# Autodesk Inventor assembly: パネル型スカラアームMISUMIアルミフレーム作成Ver
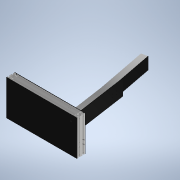
[picture p0: Inventor's stored thumbnail of the model, 180x180]
Saved by Autodesk Inventor 2022 (Build 260153000, 153)
## iProperties
Created: 2022-12-05
Part Number: パネル型スカラアームMISUMIアルミフレーム作成Ver
Document SubType Name: Assembly
Designer: tdn82
Author: tdn82
## Documents named in this file (20)
- C:\Users\tdn82\OneDrive\ドキュメント\Inventor\卒業研究パネル型スカラアーム\GrabCAD\panel-type-scalar-arm\パネル型スカラアーム\パネル型スカラアームMISUMIアルミフレーム作成Ver.iam
- C:\Users\tdn82\OneDrive\ドキュメント\Inventor\卒業研究パネル型スカラアーム\GrabCAD\panel-type-scalar-arm\パネル型スカラアーム\HFSF5-2040-180-LWH-RWH.ipt
- C:\Users\tdn82\OneDrive\ドキュメント\Inventor\卒業研究パネル型スカラアーム\GrabCAD\panel-type-scalar-arm\パネル型スカラアーム\HFSF5-2040-320-TPW.ipt
- C:\Users\tdn82\OneDrive\ドキュメント\Inventor\卒業研究パネル型スカラアーム\GrabCAD\panel-type-scalar-arm\パネル型スカラアーム\後ろカバー.ipt
- C:\Users\tdn82\OneDrive\ドキュメント\Inventor\卒業研究パネル型スカラアーム\GrabCAD\panel-type-scalar-arm\パネル型スカラアーム\サーボモータ固定用１軸目.ipt
- C:\Users\tdn82\OneDrive\ドキュメント\Inventor\卒業研究パネル型スカラアーム\GrabCAD\panel-type-scalar-arm\パネル型スカラアーム\サーボモータB3M-SC-1170-AB3M1100_scale.ipt
- C:\Users\tdn82\OneDrive\ドキュメント\Inventor\卒業研究パネル型スカラアーム\GrabCAD\panel-type-scalar-arm\パネル型スカラアーム\サーボ固定パーツ３Dプリンタ出力実験\サーボモータ固定用２軸目3mm改.ipt
- C:\Users\tdn82\OneDrive\ドキュメント\Inventor\卒業研究パネル型スカラアーム\GrabCAD\panel-type-scalar-arm\パネル型スカラアーム\横長2ndフラットバー上 アルミフレーム用.ipt
- C:\Users\tdn82\OneDrive\ドキュメント\Inventor\卒業研究パネル型スカラアーム\GrabCAD\panel-type-scalar-arm\パネル型スカラアーム\前カバー中盤左アーム固定.ipt
- C:\Users\tdn82\OneDrive\ドキュメント\Inventor\卒業研究パネル型スカラアーム\GrabCAD\panel-type-scalar-arm\パネル型スカラアーム\アルミフリーホーン02137_AluminumFreeHornWithBearing_B3M_6000.ipt
- C:\Users\tdn82\OneDrive\ドキュメント\Inventor\卒業研究パネル型スカラアーム\GrabCAD\panel-type-scalar-arm\パネル型スカラアーム\横長3rdフラットバー下.ipt
- C:\Users\tdn82\OneDrive\ドキュメント\Inventor\卒業研究パネル型スカラアーム\GrabCAD\panel-type-scalar-arm\パネル型スカラアーム\横長2ndフラットバー下 アルミフレーム用.ipt
- C:\Users\tdn82\OneDrive\ドキュメント\Inventor\卒業研究パネル型スカラアーム\GrabCAD\panel-type-scalar-arm\パネル型スカラアーム\前カバー中段右.ipt
- C:\Users\tdn82\OneDrive\ドキュメント\Inventor\卒業研究パネル型スカラアーム\GrabCAD\panel-type-scalar-arm\パネル型スカラアーム\前上カバーサーボ隠し.ipt
- C:\Users\tdn82\OneDrive\ドキュメント\Inventor\卒業研究パネル型スカラアーム\GrabCAD\panel-type-scalar-arm\パネル型スカラアーム\前下カバーサーボ隠し.ipt
- C:\Users\tdn82\OneDrive\ドキュメント\Inventor\卒業研究パネル型スカラアーム\GrabCAD\panel-type-scalar-arm\パネル型スカラアーム\ベアリング.ipt
- C:\Users\tdn82\OneDrive\ドキュメント\Inventor\卒業研究パネル型スカラアーム\GrabCAD\panel-type-scalar-arm\パネル型スカラアーム\シャフト.ipt
- C:\Users\tdn82\OneDrive\ドキュメント\Inventor\卒業研究パネル型スカラアーム\GrabCAD\panel-type-scalar-arm\パネル型スカラアーム\シャフトカラー.ipt
- C:\Users\tdn82\OneDrive\ドキュメント\Inventor\卒業研究パネル型スカラアーム\GrabCAD\panel-type-scalar-arm\パネル型スカラアーム\三段目アクリル板.ipt
- C:\Users\tdn82\OneDrive\ドキュメント\Inventor\卒業研究パネル型スカラアーム\GrabCAD\panel-type-scalar-arm\パネル型スカラアーム\シャフトカラー.iam
## Components (23 placed, 18 different names)
1. HFSF5-2040-180-LWH-RWH:1 — 挿入:6, 挿入:8, 挿入:33, 挿入:34
2. HFSF5-2040-180-LWH-RWH:2 — 挿入:5, 挿入:7, メイト:4, フラッシュ:1, メイト:12, メイト:14, メイト:26, フラッシュ:4
3. HFSF5-2040-320-TPW:1 — 挿入:5, 挿入:6, 挿入:7, 挿入:8, メイト:1, メイト:5, メイト:13
4. HFSF5-2040-320-TPW:2 — 挿入:33, 挿入:34
5. 後ろカバー:1 — メイト:1, メイト:26, フラッシュ:4
6. サーボモータ固定用１軸目:1 — 挿入:11, 挿入:12, 挿入:13, メイト:4, フラッシュ:1
7. サーボモータB3M-SC-1170-AB3M1100_scale:1 — 挿入:11, 挿入:12, 挿入:13, メイト:5, 挿入:14
8. サーボモータ固定用２軸目3mm改:1 — 挿入:15, 挿入:16, 挿入:18, 挿入:19
9. 横長2ndフラットバー上 アルミフレーム用:1 — 挿入:14, メイト:7, フラッシュ:3, メイト:19
10. 前カバー中盤左アーム固定:1 — メイト:7, 挿入:15, 挿入:16, 挿入:23, 挿入:24, フラッシュ:3, メイト:19
11. サーボモータB3M-SC-1170-AB3M1100_scale:2 — 挿入:17, 挿入:18, 挿入:19, メイト:22, 挿入:32
12. アルミフリーホーン02137_AluminumFreeHornWithBearing_B3M_6000:1 — 挿入:17, 挿入:30, 挿入:31
13. 横長3rdフラットバー下:1 — フラッシュ:2, メイト:22, 挿入:32, メイト:25
14. 横長3rdフラットバー下:2 — フラッシュ:2, 挿入:30, 挿入:31, メイト:23, メイト:24
15. 横長2ndフラットバー下 アルミフレーム用:1 — 挿入:23, 挿入:24, 挿入:26
16. 前カバー中段右:1 — メイト:12, メイト:15, メイト:16, メイト:17, メイト:18
17. 前上カバーサーボ隠し:1 — メイト:13, メイト:14, メイト:15, メイト:16
18. 前下カバーサーボ隠し:1 — メイト:17, メイト:18
19. ベアリング:1 — 挿入:26, 挿入:35
20. シャフト:1 — 挿入:36
21. シャフトカラー:2 — 挿入:35, 挿入:36, 挿入:37
22. 三段目アクリル板:1 — メイト:23, メイト:24, メイト:25
23. シャフトカラー:3 [sub-assembly] — 挿入:37
## Relationships (45: Insert 24, Mate 17, Flush 4)
- 挿入:5 [Insert]: HFSF5-2040-180-LWH-RWH:2 ↔ HFSF5-2040-320-TPW:1
- 挿入:6 [Insert]: HFSF5-2040-180-LWH-RWH:1 ↔ HFSF5-2040-320-TPW:1
- 挿入:7 [Insert]: HFSF5-2040-180-LWH-RWH:2 ↔ HFSF5-2040-320-TPW:1
- 挿入:8 [Insert]: HFSF5-2040-180-LWH-RWH:1 ↔ HFSF5-2040-320-TPW:1
- メイト:1 [Mate]: HFSF5-2040-320-TPW:1 ↔ 後ろカバー:1
- 挿入:11 [Insert]: サーボモータ固定用１軸目:1 ↔ サーボモータB3M-SC-1170-AB3M1100_scale:1
- 挿入:12 [Insert]: サーボモータ固定用１軸目:1 ↔ サーボモータB3M-SC-1170-AB3M1100_scale:1
- 挿入:13 [Insert]: サーボモータ固定用１軸目:1 ↔ サーボモータB3M-SC-1170-AB3M1100_scale:1
- メイト:4 [Mate]: HFSF5-2040-180-LWH-RWH:2 ↔ サーボモータ固定用１軸目:1
- フラッシュ:1 [Flush]: HFSF5-2040-180-LWH-RWH:2 ↔ サーボモータ固定用１軸目:1
- メイト:5 [Mate] (0.5 mm): HFSF5-2040-320-TPW:1 ↔ サーボモータB3M-SC-1170-AB3M1100_scale:1
- 挿入:14 [Insert]: サーボモータB3M-SC-1170-AB3M1100_scale:1 ↔ 横長2ndフラットバー上 アルミフレーム用:1
- メイト:7 [Mate]: 横長2ndフラットバー上 アルミフレーム用:1 ↔ 前カバー中盤左アーム固定:1
- 挿入:15 [Insert]: サーボモータ固定用２軸目3mm改:1 ↔ 前カバー中盤左アーム固定:1
- 挿入:16 [Insert]: サーボモータ固定用２軸目3mm改:1 ↔ 前カバー中盤左アーム固定:1
- 挿入:17 [Insert]: サーボモータB3M-SC-1170-AB3M1100_scale:2 ↔ アルミフリーホーン02137_AluminumFreeHornWithBearing_B3M_6000:1
- 挿入:18 [Insert]: サーボモータ固定用２軸目3mm改:1 ↔ サーボモータB3M-SC-1170-AB3M1100_scale:2
- 挿入:19 [Insert]: サーボモータ固定用２軸目3mm改:1 ↔ サーボモータB3M-SC-1170-AB3M1100_scale:2
- フラッシュ:2 [Flush]: 横長3rdフラットバー下:1 ↔ 横長3rdフラットバー下:2
- 挿入:23 [Insert]: 前カバー中盤左アーム固定:1 ↔ 横長2ndフラットバー下 アルミフレーム用:1
- 挿入:24 [Insert]: 前カバー中盤左アーム固定:1 ↔ 横長2ndフラットバー下 アルミフレーム用:1
- メイト:12 [Mate]: HFSF5-2040-180-LWH-RWH:2 ↔ 前カバー中段右:1
- メイト:13 [Mate] (-1 mm): HFSF5-2040-320-TPW:1 ↔ 前上カバーサーボ隠し:1
- メイト:14 [Mate] (-1 mm): HFSF5-2040-180-LWH-RWH:2 ↔ 前上カバーサーボ隠し:1
- メイト:15 [Mate]: 前カバー中段右:1 ↔ 前上カバーサーボ隠し:1
- メイト:16 [Mate]: 前カバー中段右:1 ↔ 前上カバーサーボ隠し:1
- メイト:17 [Mate]: 前カバー中段右:1 ↔ 前下カバーサーボ隠し:1
- メイト:18 [Mate]: 前カバー中段右:1 ↔ 前下カバーサーボ隠し:1
- フラッシュ:3 [Flush] (29 mm): 横長2ndフラットバー上 アルミフレーム用:1 ↔ 前カバー中盤左アーム固定:1
- メイト:19 [Mate]: 横長2ndフラットバー上 アルミフレーム用:1 ↔ 前カバー中盤左アーム固定:1
- 挿入:26 [Insert]: 横長2ndフラットバー下 アルミフレーム用:1 ↔ ベアリング:1
- メイト:22 [Mate]: サーボモータB3M-SC-1170-AB3M1100_scale:2 ↔ 横長3rdフラットバー下:1
- 挿入:30 [Insert]: アルミフリーホーン02137_AluminumFreeHornWithBearing_B3M_6000:1 ↔ 横長3rdフラットバー下:2
- 挿入:31 [Insert]: アルミフリーホーン02137_AluminumFreeHornWithBearing_B3M_6000:1 ↔ 横長3rdフラットバー下:2
- 挿入:32 [Insert]: サーボモータB3M-SC-1170-AB3M1100_scale:2 ↔ 横長3rdフラットバー下:1
- メイト:23 [Mate]: 横長3rdフラットバー下:2 ↔ 三段目アクリル板:1
- メイト:24 [Mate]: 横長3rdフラットバー下:2 ↔ 三段目アクリル板:1
- メイト:25 [Mate]: 横長3rdフラットバー下:1 ↔ 三段目アクリル板:1
- 挿入:33 [Insert]: HFSF5-2040-180-LWH-RWH:1 ↔ HFSF5-2040-320-TPW:2
- 挿入:34 [Insert]: HFSF5-2040-180-LWH-RWH:1 ↔ HFSF5-2040-320-TPW:2
- メイト:26 [Mate]: HFSF5-2040-180-LWH-RWH:2 ↔ 後ろカバー:1
- フラッシュ:4 [Flush]: HFSF5-2040-180-LWH-RWH:2 ↔ 後ろカバー:1
- 挿入:35 [Insert]: ベアリング:1 ↔ シャフトカラー:2
- 挿入:36 [Insert] (-5 mm): シャフト:1 ↔ シャフトカラー:2
- 挿入:37 [Insert] (2 mm): シャフトカラー:2 ↔ シャフトカラー:3
